# Autodesk Inventor assembly: Ensamblaje1168717
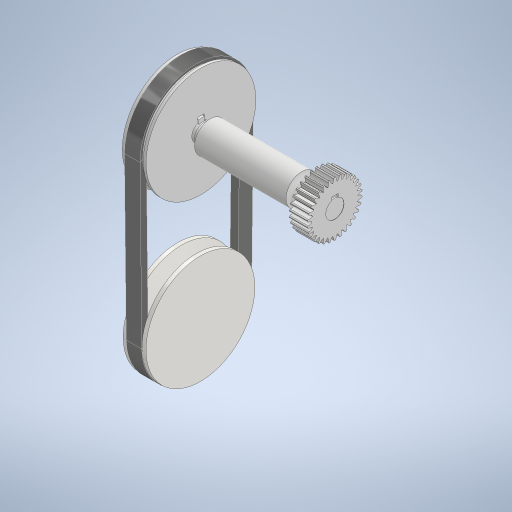
[picture p0: Inventor's stored thumbnail of the model, 512x512]
Saved by Autodesk Inventor 2024 (Build 280153000, 153)
## iProperties
Created: 2024-03-31
Part Number: Ensamblaje1168717
Document SubType Name: Assembly
Designer: mariu
Author: mariu
## Documents named in this file (6)
- C:\Users\mariu\OneDrive\Desktop\Ensamblaje1168717.iam
- C:\Users\mariu\OneDrive\Desktop\EJE_CUÑEROS.ipt
- C:\Users\mariu\OneDrive\Desktop\CUÑA.ipt
- C:\Users\mariu\Downloads\WhatsApp Unknown 2023-07-19 at 10.35.29 AM\ENGRANE.ipt
- C:\Users\mariu\OneDrive\Desktop\POLEA.ipt
- C:\Users\mariu\Downloads\WhatsApp Unknown 2023-07-19 at 10.35.29 AM\Ensamblaje1168717\Design Accelerator\Transmisión de correa trapezoidal1.iam
## Components (6 placed, 5 different names)
1. EJE_CUÑEROS:1 — Coincidencia:1, Coincidencia:2, Coincidencia:3, Coincidencia:4
2. CUÑA:1 — Coincidencia:1
3. CUÑA:2 — Coincidencia:2
4. ENGRANE:1 — Coincidencia:3
5. POLEA:1 — Coincidencia:4
6. Transmisión de correa trapezoidal:1 [sub-assembly]
## Relationships (4: Mate 4)
- Coincidencia:1 [Mate]: EJE_CUÑEROS:1 ↔ CUÑA:1
- Coincidencia:2 [Mate]: EJE_CUÑEROS:1 ↔ CUÑA:2
- Coincidencia:3 [Mate]: EJE_CUÑEROS:1 ↔ ENGRANE:1
- Coincidencia:4 [Mate]: EJE_CUÑEROS:1 ↔ POLEA:1
